# Autodesk Inventor assembly: Electronicsssssss
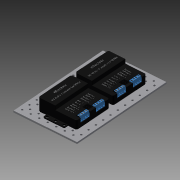
[picture p0: Inventor's stored thumbnail of the model, 180x180]
Saved by Autodesk Inventor 2014 SP2 (Build 180246200, 246)
## iProperties
Created: 2014-10-24
Part Number: Electronicsssssss
Document SubType Name: Assembly
Designer: Allison
Author: Allison
## Documents named in this file (3)
- C:\Users\Allison\Documents\inventor\InventorMasterProject\Electronicsssssss.iam
- C:\Users\Allison\Documents\Inventor\InventorMasterProject\Electronics Board.ipt
- C:\Users\Allison\Documents\Inventor\InventorMasterProject\Tetrix\Electrical\Tetrix Motor Controller.ipt
## Components (3 placed, 2 different names)
1. Electronics Board:1 — Insert:1, Insert:2, Insert:3
2. Tetrix Motor Controller:1 — Insert:1, Insert:2
3. Tetrix Motor Controller:3 — Insert:3
## Relationships (3: Insert 3)
- Insert:1: Electronics Board:1 ↔ Tetrix Motor Controller:1
- Insert:2: Electronics Board:1 ↔ Tetrix Motor Controller:1
- Insert:3: Electronics Board:1 ↔ Tetrix Motor Controller:3
